# Autodesk Inventor assembly: ASSEMBLY_Main
(part 2 of 4)
157. DIN 125-1 A A 3,2:54 — Mate:569, Mate:570, Insert:151
158. DIN 934 - replaced by DIN EN 24032/28673/28674 M3:16 — Insert:154
159. DIN 125-1 A A 3,2:53 — Mate:575, Mate:576, Insert:154
160. DIN 912 - replaced by DIN EN ISO 4762 M3 x 16:5 — Insert:150
161. DIN 125-1 A A 3,2:52 — Mate:567, Mate:568, Insert:150
162. DIN 934 - replaced by DIN EN 24032/28673/28674 M3:15 — Insert:149
163. DIN 125-1 A A 3,2:51 — Mate:565, Mate:566, Insert:149
164. DIN 912 - replaced by DIN EN ISO 4762 M3 x 10:4 — Insert:147
165. DIN 125-1 A A 3,2:50 — Mate:561, Mate:562, Insert:147
166. DIN 934 - replaced by DIN EN 24032/28673/28674 M3:14 — Insert:148
167. DIN 125-1 A A 3,2:49 — Mate:563, Mate:564, Insert:148
168. DIN 125-1 A A 5,3:51 — Mate:481, Mate:482, Insert:107
169. DIN 125-1 A A 5,3:92 — Mate:603, Mate:604, Insert:168
170. DIN 912 - replaced by DIN EN ISO 4762 M5 x 10:29 — Insert:167
171. DIN 125-1 A A 5,3:91 — Mate:601, Mate:602, Insert:167
172. DIN 912 - replaced by DIN EN ISO 4762 M5 x 10:28 — Insert:166
173. DIN 912 - replaced by DIN EN ISO 4762 M5 x 10:27 — Insert:165
174. DIN 912 - replaced by DIN EN ISO 4762 M5 x 10:26 — Insert:164
175. DIN 125-1 A A 5,3:90 — Mate:599, Mate:600, Insert:166
176. DIN 125-1 A A 5,3:89 — Mate:597, Mate:598, Insert:165
177. DIN 125-1 A A 5,3:88 — Mate:595, Mate:596, Insert:164
178. DIN 912 - replaced by DIN EN ISO 4762 M5 x 10:25 — Insert:163
179. DIN 125-1 A A 5,3:87 — Mate:593, Mate:594, Insert:163
180. DIN 912 - replaced by DIN EN ISO 4762 M5 x 8:25 — Insert:162
181. DIN 125-1 A A 5,3:86 — Mate:591, Mate:592, Insert:162
182. DIN 912 - replaced by DIN EN ISO 4762 M5 x 12:12 — Insert:161
183. DIN 125-1 A A 5,3:85 — Mate:589, Mate:590, Insert:161
184. DIN 912 - replaced by DIN EN ISO 4762 M5 x 12:11 — Insert:160
185. DIN 125-1 A A 5,3:84 — Mate:587, Mate:588, Insert:160
186. DIN 912 - replaced by DIN EN ISO 4762 M5 x 8:24 — Insert:159
187. DIN 125-1 A A 5,3:83 — Mate:585, Mate:586, Insert:159
188. DIN 912 - replaced by DIN EN ISO 4762 M5 x 8:23 — Insert:158
189. DIN 125-1 A A 5,3:82 — Mate:583, Mate:584, Insert:158
190. DIN 934 - replaced by DIN EN 24032/28673/28674 M3:19 — Insert:157
191. DIN 934 - replaced by DIN EN 24032/28673/28674 M3:18 — Insert:156
192. DIN 934 - replaced by DIN EN 24032/28673/28674 M3:17 — Insert:155
193. DIN 912 - replaced by DIN EN ISO 4762 M3 x 10:3 — Insert:146
194. DIN 125-1 A A 3,2:48 — Mate:559, Mate:560, Insert:146
195. DIN 934 - replaced by DIN EN 24032/28673/28674 M3:13 — Insert:145
196. DIN 125-1 A A 3,2:47 — Mate:557, Mate:558, Insert:145
197. DIN 912 - replaced by DIN EN ISO 4762 M3 x 10:2 — Insert:143
198. DIN 125-1 A A 3,2:46 — Mate:553, Mate:554, Insert:143
199. DIN 934 - replaced by DIN EN 24032/28673/28674 M3:12 — Insert:144
200. DIN 125-1 A A 3,2:45 — Mate:555, Mate:556, Insert:144
201. DIN 912 - replaced by DIN EN ISO 4762 M3 x 10:1 — Insert:142
202. DIN 125-1 A A 3,2:44 — Mate:551, Mate:552, Insert:142
203. DIN 912 - replaced by DIN EN ISO 4762 M5 x 30:13 — Insert:141
204. DIN 125-1 A A 5,3:81 — Mate:549, Mate:550, Insert:141
205. DIN 912 - replaced by DIN EN ISO 4762 M5 x 8:22 — Insert:140
206. DIN 125-1 A A 5,3:80 — Mate:547, Mate:548, Insert:140
207. DIN 912 - replaced by DIN EN ISO 4762 M5 x 8:21 — Insert:139
208. DIN 125-1 A A 5,3:79 — Mate:545, Mate:546, Insert:139
209. DIN 912 - replaced by DIN EN ISO 4762 M5 x 10:24 — Insert:138
210. DIN 912 - replaced by DIN EN ISO 4762 M5 x 10:23 — Insert:137
211. DIN 912 - replaced by DIN EN ISO 4762 M5 x 10:22 — Insert:136
212. DIN 125-1 A A 5,3:78 — Mate:543, Mate:544, Insert:138
213. DIN 125-1 A A 5,3:77 — Mate:541, Mate:542, Insert:137
214. DIN 125-1 A A 5,3:76 — Mate:539, Mate:540, Insert:136
215. DIN 912 - replaced by DIN EN ISO 4762 M5 x 10:21 — Insert:135
216. DIN 125-1 A A 5,3:75 — Mate:537, Mate:538, Insert:135
217. DIN 912 - replaced by DIN EN ISO 4762 M5 x 10:20 — Insert:134
218. DIN 912 - replaced by DIN EN ISO 4762 M5 x 10:19 — Insert:133
219. DIN 912 - replaced by DIN EN ISO 4762 M5 x 10:18 — Insert:132
220. DIN 125-1 A A 5,3:74 — Mate:535, Mate:536, Insert:134
221. DIN 125-1 A A 5,3:73 — Mate:533, Mate:534, Insert:133
222. DIN 125-1 A A 5,3:72 — Mate:531, Mate:532, Insert:132
223. DIN 912 - replaced by DIN EN ISO 4762 M5 x 10:17 — Insert:131
224. DIN 125-1 A A 5,3:71 — Mate:529, Mate:530, Insert:131
225. DIN 912 - replaced by DIN EN ISO 4762 M5 x 10:16 — Insert:130
226. DIN 125-1 A A 5,3:70 — Mate:527, Mate:528, Insert:130
227. DIN 912 - replaced by DIN EN ISO 4762 M5 x 10:15 — Insert:129
228. DIN 125-1 A A 5,3:69 — Mate:525, Mate:526, Insert:129
229. DIN 912 - replaced by DIN EN ISO 4762 M5 x 10:14 — Insert:128
230. DIN 125-1 A A 5,3:68 — Mate:523, Mate:524, Insert:128
231. DIN 912 - replaced by DIN EN ISO 4762 M5 x 10:13 — Insert:127
232. DIN 125-1 A A 5,3:67 — Mate:521, Mate:522, Insert:127
233. DIN 912 - replaced by DIN EN ISO 4762 M4 x 10:4 — Insert:126
234. DIN 912 - replaced by DIN EN ISO 4762 M4 x 10:3 — Insert:125
235. DIN 912 - replaced by DIN EN ISO 4762 M4 x 10:2 — Insert:124
236. DIN 125-1 A A 4,3:20 — Mate:519, Mate:520, Insert:126
237. DIN 125-1 A A 4,3:19 — Mate:517, Mate:518, Insert:125
238. DIN 125-1 A A 4,3:18 — Mate:515, Mate:516, Insert:124
239. DIN 912 - replaced by DIN EN ISO 4762 M4 x 10:1 — Insert:123
240. DIN 125-1 A A 4,3:17 — Mate:513, Mate:514, Insert:123
241. DIN 912 - replaced by DIN EN ISO 4762 M4 x 8:4 — Insert:122
242. DIN 912 - replaced by DIN EN ISO 4762 M4 x 8:3 — Insert:121
243. DIN 912 - replaced by DIN EN ISO 4762 M4 x 8:2 — Insert:120
244. DIN 125-1 A A 4,3:16 — Mate:511, Mate:512, Insert:122
245. DIN 125-1 A A 4,3:15 — Mate:509, Mate:510, Insert:121
246. DIN 125-1 A A 4,3:14 — Mate:507, Mate:508, Insert:120
247. DIN 912 - replaced by DIN EN ISO 4762 M4 x 8:1 — Insert:119
248. DIN 125-1 A A 4,3:13 — Mate:505, Mate:506, Insert:119
249. DIN 912 - replaced by DIN EN ISO 4762 M5 x 10:12 — Insert:118
250. DIN 125-1 A A 5,3:66 — Mate:503, Mate:504, Insert:118
251. DIN 912 - replaced by DIN EN ISO 4762 M5 x 10:11 — Insert:117
252. DIN 125-1 A A 5,3:65 — Mate:501, Mate:502, Insert:117
253. DIN 912 - replaced by DIN EN ISO 4762 M5 x 10:10 — Insert:116
254. DIN 125-1 A A 5,3:64 — Mate:499, Mate:500, Insert:116
255. DIN 912 - replaced by DIN EN ISO 4762 M5 x 10:9 — Insert:115
256. DIN 125-1 A A 5,3:63 — Mate:497, Mate:498, Insert:115
257. DIN 912 - replaced by DIN EN ISO 4762 M5 x 12:10 — Insert:114
258. DIN 125-1 A A 5,3:62 — Mate:495, Mate:496, Insert:114
259. DIN 912 - replaced by DIN EN ISO 4762 M5 x 12:9 — Insert:113
260. DIN 125-1 A A 5,3:61 — Mate:493, Mate:494, Insert:113
261. DIN 912 - replaced by DIN EN ISO 4762 M5 x 12:8 — Insert:112
262. DIN 125-1 A A 5,3:60 — Mate:491, Mate:492, Insert:112
263. DIN 912 - replaced by DIN EN ISO 4762 M5 x 12:7 — Insert:111
264. DIN 125-1 A A 5,3:59 — Mate:489, Mate:490, Insert:111
265. DIN 912 - replaced by DIN EN ISO 4762 M5 x 10:8 — Insert:110
266. DIN 125-1 A A 5,3:58 — Mate:487, Mate:488, Insert:110
267. DIN 912 - replaced by DIN EN ISO 4762 M5 x 10:7 — Insert:109
268. DIN 125-1 A A 5,3:57 — Mate:485, Mate:486, Insert:109
269. DIN 912 - replaced by DIN EN ISO 4762 M5 x 10:6 — Insert:108
270. DIN 125-1 A A 5,3:52 — Mate:483, Mate:484, Insert:108
271. DIN 912 - replaced by DIN EN ISO 4762 M5 x 10:5 — Insert:107
272. DIN 912 - replaced by DIN EN ISO 4762 M5 x 10:2 — Insert:106
273. DIN 125-1 A A 5,3:50 — Mate:479, Mate:480, Insert:106
274. DIN 912 - replaced by DIN EN ISO 4762 M5 x 10:1 — Insert:105
275. DIN 125-1 A A 5,3:49 — Mate:477, Mate:478, Insert:105
276. DIN 912 - replaced by DIN EN ISO 4762 M5 x 12:5 — Insert:104
277. DIN 125-1 A A 5,3:53 — Mate:475, Mate:476, Insert:104
278. DIN 912 - replaced by DIN EN ISO 4762 M5 x 12:6 — Insert:103
279. DIN 125-1 A A 5,3:54 — Mate:473, Mate:474, Insert:103
280. DIN 912 - replaced by DIN EN ISO 4762 M5 x 10:3 — Insert:102
281. DIN 125-1 A A 5,3:55 — Mate:471, Mate:472, Insert:102
282. DIN 912 - replaced by DIN EN ISO 4762 M5 x 10:4 — Insert:101
283. DIN 125-1 A A 5,3:56 — Mate:469, Mate:470, Insert:101
284. DIN 912 - replaced by DIN EN ISO 4762 M3 x 8:2 — Insert:66
285. DIN 125-1 A A 3,2:17 — Mate:387, Mate:388, Insert:66
286. DIN 912 - replaced by DIN EN ISO 4762 M3 x 8:1 — Insert:65
287. DIN 125-1 A A 3,2:16 — Mate:385, Mate:386, Insert:65
288. DIN 125-1 A A 3,2:30 — Mate:423, Mate:424, Insert:79
289. DIN 125-1 A A 3,2:29 — Mate:421, Mate:422, Insert:78
290. ISO 7380-1 M3 x 20:9 — Insert:76
291. ISO 7380-1 M3 x 20:8 — Insert:75
292. ISO 7380-1 M3 x 20:7 — Insert:74
293. ISO 7380-1 M3 x 20:6 — Insert:73
294. ISO 7380-1 M3 x 20:5 — Insert:72
295. ISO 7380-1 M3 x 20:4 — Insert:71
296. ISO 7380-1 M3 x 20:3 — Insert:70
297. DIN 125-1 A A 3,2:28 — Mate:417, Mate:418, Insert:76
298. DIN 125-1 A A 3,2:27 — Mate:415, Mate:416, Insert:75
299. DIN 125-1 A A 3,2:26 — Mate:413, Mate:414, Insert:74
300. DIN 125-1 A A 3,2:25 — Mate:411, Mate:412, Insert:73
301. DIN 125-1 A A 3,2:24 — Mate:409, Mate:410, Insert:72
302. DIN 125-1 A A 3,2:23 — Mate:407, Mate:408, Insert:71
303. DIN 125-1 A A 3,2:22 — Mate:405, Mate:406, Insert:70
304. DIN 934 - replaced by DIN EN 24032/28673/28674 M3:4 — Insert:77
305. DIN 125-1 A A 3,2:21 — Mate:419, Mate:420, Insert:77
306. ISO 7380-1 M3 x 20:2 — Insert:69
307. DIN 125-1 A A 3,2:20 — Mate:403, Mate:404, Insert:69
308. DIN 7991 M3x8:2 — Mate:402
309. DIN 7991 M3x8:1 — Mate:401
310. DIN 912 - replaced by DIN EN ISO 4762 M3 x 8:4 — Insert:68
311. DIN 125-1 A A 3,2:19 — Mate:393, Mate:394, Insert:68
312. DIN 912 - replaced by DIN EN ISO 4762 M3 x 8:3 — Insert:67
313. DIN 125-1 A A 3,2:18 — Mate:391, Mate:392, Insert:67
314. DIN 125-1 A A 3,2:43 — Mate:451, Mate:452, Insert:92
315. DIN 125-1 A A 3,2:42 — Mate:449, Mate:450, Insert:91
316. DIN 125-1 A A 3,2:41 — Mate:447, Mate:448, Insert:90
317. DIN 125-1 A A 3,2:40 — Mate:445, Mate:446, Insert:89
318. DIN 125-1 A A 3,2:39 — Mate:443, Mate:444, Insert:88
319. DIN 125-1 A A 3,2:38 — Mate:441, Mate:442, Insert:87
320. DIN 125-1 A A 3,2:37 — Mate:439, Mate:440, Insert:86
321. DIN 912 - replaced by DIN EN ISO 4762 M3 x 8:5 — Insert:85
322. DIN 125-1 A A 3,2:36 — Mate:437, Mate:438, Insert:85
323. DIN 934 - replaced by DIN EN 24032/28673/28674 M3:11 — Insert:84
324. DIN 934 - replaced by DIN EN 24032/28673/28674 M3:10 — Insert:83
325. DIN 934 - replaced by DIN EN 24032/28673/28674 M3:9 — Insert:82
326. DIN 934 - replaced by DIN EN 24032/28673/28674 M3:8 — Insert:81
327. DIN 934 - replaced by DIN EN 24032/28673/28674 M3:7 — Insert:80
328. DIN 934 - replaced by DIN EN 24032/28673/28674 M3:6 — Insert:79
329. DIN 934 - replaced by DIN EN 24032/28673/28674 M3:5 — Insert:78
330. DIN 125-1 A A 3,2:35 — Mate:433, Mate:434, Insert:84
331. DIN 125-1 A A 3,2:34 — Mate:431, Mate:432, Insert:83
332. DIN 125-1 A A 3,2:33 — Mate:429, Mate:430, Insert:82
333. DIN 125-1 A A 3,2:32 — Mate:427, Mate:428, Insert:81
334. DIN 125-1 A A 3,2:31 — Mate:425, Mate:426, Insert:80
335. DIN 934 - replaced by DIN EN 24032/28673/28674 M4:6 — Insert:100
336. DIN 934 - replaced by DIN EN 24032/28673/28674 M4:5 — Insert:99
337. DIN 934 - replaced by DIN EN 24032/28673/28674 M4:4 — Insert:98
338. DIN 125-1 A A 4,3:12 — Mate:467, Mate:468, Insert:100
339. DIN 125-1 A A 4,3:11 — Mate:465, Mate:466, Insert:99
340. DIN 125-1 A A 4,3:10 — Mate:463, Mate:464, Insert:98
341. DIN 912 - replaced by DIN EN ISO 4762 M4 x 40:4 — Insert:96
342. DIN 912 - replaced by DIN EN ISO 4762 M4 x 40:3 — Insert:95
343. DIN 912 - replaced by DIN EN ISO 4762 M4 x 40:2 — Insert:94
344. DIN 125-1 A A 4,3:9 — Mate:459, Mate:460, Insert:96
345. DIN 125-1 A A 4,3:8 — Mate:457, Mate:458, Insert:95
346. DIN 125-1 A A 4,3:7 — Mate:455, Mate:456, Insert:94
347. DIN 934 - replaced by DIN EN 24032/28673/28674 M4:3 — Insert:97
348. DIN 125-1 A A 4,3:6 — Mate:461, Mate:462, Insert:97
349. DIN 912 - replaced by DIN EN ISO 4762 M4 x 40:1 — Insert:93
350. DIN 125-1 A A 4,3:5 — Mate:453, Mate:454, Insert:93
351. DIN 912 - replaced by DIN EN ISO 4762 M3 x 8:12 — Insert:92
352. DIN 912 - replaced by DIN EN ISO 4762 M3 x 8:11 — Insert:91
353. DIN 912 - replaced by DIN EN ISO 4762 M3 x 8:10 — Insert:90
354. DIN 912 - replaced by DIN EN ISO 4762 M3 x 8:9 — Insert:89
355. DIN 912 - replaced by DIN EN ISO 4762 M3 x 8:8 — Insert:88
356. DIN 912 - replaced by DIN EN ISO 4762 M3 x 8:7 — Insert:87
357. DIN 912 - replaced by DIN EN ISO 4762 M3 x 8:6 — Insert:86
358. DIN 912 - replaced by DIN EN ISO 4762 M5 x 8:5 — Insert:45
359. DIN 912 - replaced by DIN EN ISO 4762 M5 x 8:4 — Insert:44
360. DIN 912 - replaced by DIN EN ISO 4762 M5 x 8:3 — Insert:43
361. DIN 912 - replaced by DIN EN ISO 4762 M5 x 8:2 — Insert:42
362. DIN 125-1 A A 5,3:29 — Mate:336, Mate:337, Insert:45
363. DIN 125-1 A A 5,3:28 — Mate:334, Mate:335, Insert:44
364. DIN 125-1 A A 5,3:27 — Mate:332, Mate:333, Insert:43
365. DIN 125-1 A A 5,3:26 — Mate:330, Mate:331, Insert:42
366. DIN 912 - replaced by DIN EN ISO 4762 M5 x 8:1 — Insert:41
367. DIN 125-1 A A 5,3:25 — Mate:328, Mate:329, Insert:41
368. DIN 934 - replaced by DIN EN 24032/28673/28674 M5:4 — Insert:40
369. DIN 125-1 A A 5,3:24 — Mate:326, Mate:327, Insert:40
370. DIN 912 - replaced by DIN EN ISO 4762 M5 x 25:4 — Insert:38
371. DIN 125-1 A A 5,3:23 — Mate:322, Mate:323, Insert:38
372. DIN 934 - replaced by DIN EN 24032/28673/28674 M5:3 — Insert:39
373. DIN 125-1 A A 5,3:22 — Mate:324, Mate:325, Insert:39
374. DIN 912 - replaced by DIN EN ISO 4762 M5 x 25:3 — Insert:37
375. DIN 125-1 A A 5,3:21 — Mate:320, Mate:321, Insert:37
376. DIN 934 - replaced by DIN EN 24032/28673/28674 M5:2 — Insert:36
377. DIN 125-1 A A 5,3:20 — Mate:318, Mate:319, Insert:36
378. DIN 912 - replaced by DIN EN ISO 4762 M5 x 25:2 — Insert:34
379. DIN 125-1 A A 5,3:19 — Mate:314, Mate:315, Insert:34
380. DIN 934 - replaced by DIN EN 24032/28673/28674 M5:1 — Insert:35
381. DIN 125-1 A A 5,3:18 — Mate:316, Mate:317, Insert:35
382. DIN 912 - replaced by DIN EN ISO 4762 M5 x 25:1 — Insert:33
383. DIN 125-1 A A 5,3:17 — Mate:312, Mate:313, Insert:33
384. DIN 912 - replaced by DIN EN ISO 4762 M5 x 8:10 — Insert:50
385. DIN 912 - replaced by DIN EN ISO 4762 M5 x 8:9 — Insert:49
386. DIN 912 - replaced by DIN EN ISO 4762 M5 x 8:8 — Insert:48
387. DIN 912 - replaced by DIN EN ISO 4762 M5 x 8:7 — Insert:47
388. DIN 125-1 A A 5,3:34 — Insert:50
389. DIN 125-1 A A 5,3:33 — Insert:49
390. DIN 125-1 A A 5,3:32 — Insert:48
391. DIN 125-1 A A 5,3:31 — Insert:47
392. DIN 912 - replaced by DIN EN ISO 4762 M5 x 8:6 — Insert:46
393. DIN 125-1 A A 5,3:30 — Insert:46
394. DIN 912 - replaced by DIN EN ISO 4762 M5 x 8:15 — Insert:55
395. DIN 912 - replaced by DIN EN ISO 4762 M5 x 8:14 — Insert:54
396. DIN 912 - replaced by DIN EN ISO 4762 M5 x 8:13 — Insert:53
397. DIN 912 - replaced by DIN EN ISO 4762 M5 x 8:12 — Insert:52
398. DIN 125-1 A A 5,3:39 — Insert:55
399. DIN 125-1 A A 5,3:38 — Insert:54
400. DIN 125-1 A A 5,3:37 — Insert:53
401. DIN 125-1 A A 5,3:36 — Insert:52
402. DIN 912 - replaced by DIN EN ISO 4762 M5 x 8:11 — Insert:51
403. DIN 125-1 A A 5,3:35 — Insert:51
404. DIN 912 - replaced by DIN EN ISO 4762 M5 x 12:4 — Insert:64
405. DIN 912 - replaced by DIN EN ISO 4762 M5 x 12:3 — Insert:63
406. DIN 912 - replaced by DIN EN ISO 4762 M5 x 12:2 — Insert:62
407. DIN 125-1 A A 5,3:48 — Mate:371, Mate:372, Insert:64
408. DIN 125-1 A A 5,3:47 — Mate:369, Mate:370, Insert:63
409. DIN 125-1 A A 5,3:46 — Mate:367, Mate:368, Insert:62
410. DIN 912 - replaced by DIN EN ISO 4762 M5 x 12:1 — Insert:61
411. DIN 125-1 A A 5,3:45 — Mate:365, Mate:366, Insert:61
412. DIN 912 - replaced by DIN EN ISO 4762 M5 x 8:20 — Insert:60
413. DIN 912 - replaced by DIN EN ISO 4762 M5 x 8:19 — Insert:59
414. DIN 912 - replaced by DIN EN ISO 4762 M5 x 8:18 — Insert:58
415. DIN 912 - replaced by DIN EN ISO 4762 M5 x 8:17 — Insert:57
416. DIN 125-1 A A 5,3:44 — Insert:60
417. DIN 125-1 A A 5,3:43 — Insert:59
418. DIN 125-1 A A 5,3:42 — Insert:58
419. DIN 125-1 A A 5,3:41 — Insert:57
420. DIN 912 - replaced by DIN EN ISO 4762 M5 x 8:16 — Insert:56
421. DIN 125-1 A A 5,3:40 — Insert:56
422. DIN 934 - replaced by DIN EN 24032/28673/28674 M4:2 — Insert:31
423. DIN 125-1 A A 4,3:4 — Mate:304, Mate:305, Insert:31
424. DIN 912 - replaced by DIN EN ISO 4762 M4 x 30:2 — Insert:29
425. DIN 125-1 A A 4,3:3 — Mate:300, Mate:301, Insert:29
426. DIN 934 - replaced by DIN EN 24032/28673/28674 M4:1 — Insert:30
427. DIN 125-1 A A 4,3:2 — Mate:302, Mate:303, Insert:30
428. DIN 912 - replaced by DIN EN ISO 4762 M4 x 30:1 — Insert:28
429. DIN 125-1 A A 4,3:1 — Mate:298, Mate:299, Insert:28
430. DIN 934 - replaced by DIN EN 24032/28673/28674 M3:3 — Insert:27
431. DIN 125-1 A A 3,2:11 — Mate:296, Mate:297, Insert:27
432. DIN 912 - replaced by DIN EN ISO 4762 M3 x 20:1 — Insert:26
433. DIN 125-1 A A 3,2:10 — Mate:294, Mate:295, Insert:26
434. DIN 934 - replaced by DIN EN 24032/28673/28674 M3:2 — Insert:25
435. DIN 125-1 A A 3,2:9 — Mate:292, Mate:293, Insert:25
436. ISO 7380-1 M3 x 20:1 — Insert:24
437. DIN 125-1 A A 3,2:8 — Mate:290, Mate:291, Insert:24
438. DIN 934 - replaced by DIN EN 24032/28673/28674 M3:1 — Insert:23
439. DIN 125-1 A A 3,2:7 — Mate:288, Mate:289, Insert:23
440. ISO 7380-1 M3 x 30:1 — Insert:22
441. DIN 125-1 A A 3,2:6 — Mate:286, Mate:287, Insert:22
442. ISO 7380-1 M3 x 12:5 — Insert:21
443. ISO 7380-1 M3 x 12:4 — Insert:20
444. ISO 7380-1 M3 x 12:3 — Insert:19
445. ISO 7380-1 M3 x 12:2 — Insert:18
446. DIN 125-1 A A 3,2:5 — Mate:284, Mate:285, Insert:21
447. DIN 125-1 A A 3,2:4 — Mate:282, Mate:283, Insert:20
448. DIN 125-1 A A 3,2:3 — Mate:280, Mate:281, Insert:19
449. DIN 125-1 A A 3,2:2 — Mate:278, Mate:279, Insert:18
450. ISO 7380-1 M3 x 12:1 — Insert:17
451. DIN 125-1 A A 3,2:1 — Mate:276, Mate:277, Insert:17
452. DIN 912 - replaced by DIN EN ISO 4762 M5 x 50:4 — Insert:16
453. DIN 912 - replaced by DIN EN ISO 4762 M5 x 50:3 — Insert:15
454. DIN 912 - replaced by DIN EN ISO 4762 M5 x 50:2 — Insert:14
455. DIN 125-1 A A 5,3:16 — Mate:274, Mate:275, Insert:16
456. DIN 125-1 A A 5,3:15 — Mate:272, Mate:273, Insert:15
457. DIN 125-1 A A 5,3:14 — Mate:270, Mate:271, Insert:14
458. DIN 912 - replaced by DIN EN ISO 4762 M5 x 50:1 — Insert:13
459. DIN 125-1 A A 5,3:13 — Mate:268, Mate:269, Insert:13
460. DIN 912 - replaced by DIN EN ISO 4762 M5 x 30:12 — Insert:12
461. DIN 912 - replaced by DIN EN ISO 4762 M5 x 30:11 — Insert:11
462. DIN 912 - replaced by DIN EN ISO 4762 M5 x 30:10 — Insert:10
463. DIN 912 - replaced by DIN EN ISO 4762 M5 x 30:9 — Insert:9
464. DIN 912 - replaced by DIN EN ISO 4762 M5 x 30:8 — Insert:8
465. DIN 912 - replaced by DIN EN ISO 4762 M5 x 30:7 — Insert:7
466. DIN 912 - replaced by DIN EN ISO 4762 M5 x 30:6 — Insert:6
467. DIN 912 - replaced by DIN EN ISO 4762 M5 x 30:5 — Insert:5
468. DIN 912 - replaced by DIN EN ISO 4762 M5 x 30:4 — Insert:4
469. DIN 912 - replaced by DIN EN ISO 4762 M5 x 30:3 — Insert:3
470. DIN 912 - replaced by DIN EN ISO 4762 M5 x 30:2 — Insert:2
471. DIN 125-1 A A 5,3:12 — Mate:266, Mate:267, Insert:12
472. DIN 125-1 A A 5,3:11 — Mate:264, Mate:265, Insert:11
473. DIN 125-1 A A 5,3:10 — Mate:262, Mate:263, Insert:10
474. DIN 125-1 A A 5,3:9 — Mate:260, Mate:261, Insert:9
475. DIN 125-1 A A 5,3:8 — Mate:258, Mate:259, Insert:8
476. DIN 125-1 A A 5,3:7 — Mate:256, Mate:257, Insert:7
477. DIN 125-1 A A 5,3:6 — Mate:254, Mate:255, Insert:6
478. DIN 125-1 A A 5,3:5 — Mate:252, Mate:253, Insert:5
479. DIN 125-1 A A 5,3:4 — Mate:250, Mate:251, Insert:4
480. DIN 125-1 A A 5,3:3 — Mate:248, Mate:249, Insert:3
481. DIN 125-1 A A 5,3:2 — Mate:246, Mate:247, Insert:2
482. DIN 912 - replaced by DIN EN ISO 4762 M5 x 30:1 — Insert:1
483. DIN 125-1 A A 5,3:1 — Mate:244, Mate:245, Insert:1
484. ISO 10642 M4x20:1 — Mate:641, Mate:642
485. DIN 934 - replaced by DIN EN 24032/28673/28674 M4:8 — Insert:172
486. DIN 934 - replaced by DIN EN 24032/28673/28674 M4:7 — Insert:171
487. ISO 10642 M4x20:2
488. DIN 934 - replaced by DIN EN 24032/28673/28674 M4:9
489. DIN 934 - replaced by DIN EN 24032/28673/28674 M4:10
490. ISO 10642 M4x20:3
491. DIN 934 - replaced by DIN EN 24032/28673/28674 M4:11
492. DIN 934 - replaced by DIN EN 24032/28673/28674 M4:12
493. ISO 10642 M4x20:4
494. DIN 934 - replaced by DIN EN 24032/28673/28674 M4:13
495. DIN 934 - replaced by DIN EN 24032/28673/28674 M4:14
496. DIN 912 - replaced by DIN EN ISO 4762 M3 x 16:1 — Insert:32, Mate:310
497. DIN 125-1 A A 3,2:12 — Mate:308, Mate:309, Insert:32
498. COTS_GENERIC_20x20_M3_Nut:1 — Mate:306, Mate:307, Mate:310
499. DIN 912 - replaced by DIN EN ISO 4762 M3 x 16:2
500. DIN 125-1 A A 3,2:13
501. COTS_GENERIC_20x20_M3_Nut:2
502. DIN 912 - replaced by DIN EN ISO 4762 M3 x 16:3
503. DIN 125-1 A A 3,2:14
504. COTS_GENERIC_20x20_M3_Nut:3
505. DIN 912 - replaced by DIN EN ISO 4762 M3 x 16:4
506. DIN 125-1 A A 3,2:15
507. COTS_GENERIC_20x20_M3_Nut:4
## Component patterns: (2 elements), (4 elements, first: ISO 10642 M4x20:1 + DIN 934 - replaced by DIN EN 24032/28673/28674 M4:8 + DIN 934 - replaced by DIN EN 24032/28673/28674 M4:7), (2 elements, first: DIN 912 - replaced by DIN EN ISO 4762 M3 x 16:1 + DIN 125-1 A A 3,2:12 + COTS_GENERIC_20x20_M3_Nut:1), Component Pattern 1:2 (2 elements)
## Relationships (862: Mate 549, Insert 172, Flush 139, Angle 2)
- Zestawiający:7 [Mate]: COTS_GENERIC_20x40mm_alu_extrusion_460mm:1 ↔ COTS_GENERIC_20x40mm_alu_extrusion_560mm:1
- Równoległy:13 [Flush]: COTS_GENERIC_20x40mm_alu_extrusion_460mm:1 ↔ COTS_GENERIC_20x40mm_alu_extrusion_560mm:1
- Równoległy:14 [Flush]: COTS_GENERIC_20x40mm_alu_extrusion_460mm:1 ↔ COTS_GENERIC_20x40mm_alu_extrusion_560mm:1
- Zestawiający:8 [Mate]: COTS_GENERIC_20x40mm_alu_extrusion_460mm:2 ↔ COTS_GENERIC_20x40mm_alu_extrusion_560mm:1
- Równoległy:15 [Flush]: COTS_GENERIC_20x40mm_alu_extrusion_460mm:2 ↔ COTS_GENERIC_20x40mm_alu_extrusion_560mm:1
- Równoległy:16 [Flush]: COTS_GENERIC_20x40mm_alu_extrusion_460mm:2 ↔ COTS_GENERIC_20x40mm_alu_extrusion_560mm:1
- Zestawiający:9 [Mate]: COTS_GENERIC_20x40mm_alu_extrusion_460mm:1 ↔ COTS_GENERIC_20x40mm_alu_extrusion_560mm:3
- Równoległy:17 [Flush]: COTS_GENERIC_20x40mm_alu_extrusion_460mm:1 ↔ COTS_GENERIC_20x40mm_alu_extrusion_560mm:3
- Równoległy:18 [Flush]: COTS_GENERIC_20x40mm_alu_extrusion_460mm:1 ↔ COTS_GENERIC_20x40mm_alu_extrusion_560mm:3
- Zestawiający:10 [Mate]: COTS_GENERIC_20x40mm_alu_extrusion_460mm:1 ↔ COTS_GENERIC_20x40mm_alu_extrusion_460mm:3
- Równoległy:19 [Flush]: COTS_GENERIC_20x40mm_alu_extrusion_460mm:1 ↔ COTS_GENERIC_20x40mm_alu_extrusion_460mm:3
- Zestawiający:11 [Mate]: COTS_GENERIC_20x40mm_alu_extrusion_460mm:2 ↔ COTS_GENERIC_20x40mm_alu_extrusion_460mm:4
- Równoległy:20 [Flush]: COTS_GENERIC_20x40mm_alu_extrusion_460mm:2 ↔ COTS_GENERIC_20x40mm_alu_extrusion_460mm:4
- Zestawiający:12 [Mate]: COTS_GENERIC_20x40mm_alu_extrusion_460mm:3 ↔ COTS_GENERIC_20x40mm_alu_extrusion_560mm:2
- Równoległy:21 [Flush]: COTS_GENERIC_20x40mm_alu_extrusion_460mm:3 ↔ COTS_GENERIC_20x40mm_alu_extrusion_560mm:2
- Równoległy:22 [Flush]: COTS_GENERIC_20x40mm_alu_extrusion_460mm:3 ↔ COTS_GENERIC_20x40mm_alu_extrusion_560mm:2
- Równoległy:23 [Flush]: COTS_GENERIC_20x40mm_alu_extrusion_460mm:4 ↔ COTS_GENERIC_20x40mm_alu_extrusion_560mm:2
- Równoległy:24 [Flush]: COTS_GENERIC_20x40mm_alu_extrusion_460mm:4 ↔ COTS_GENERIC_20x40mm_alu_extrusion_560mm:2
- Równoległy:25 [Flush] (156.5 mm): COTS_GENERIC_20x40mm_alu_extrusion_460mm:1 ↔ COTS_GENERIC_20x40mm_alu_extrusion_460mm:3
- Zestawiający:13 [Mate]: COTS_GENERIC_20x40mm_alu_extrusion_460mm:3 ↔ LC_ALU_3mm_Top_Beam_Mounting_Bracket:1
- Zestawiający:14 [Mate]: COTS_GENERIC_20x40mm_alu_extrusion_560mm:2 ↔ LC_ALU_3mm_Top_Beam_Mounting_Bracket:2
- Zestawiający:15 [Mate]: COTS_GENERIC_20x40mm_alu_extrusion_560mm:2 ↔ LC_ALU_3mm_Top_Beam_Mounting_Bracket:3
- Zestawiający:16 [Mate]: COTS_GENERIC_20x40mm_alu_extrusion_460mm:4 ↔ LC_ALU_3mm_Top_Beam_Mounting_Bracket:4
- Równoległy:26 [Flush]: COTS_GENERIC_20x40mm_alu_extrusion_460mm:3 ↔ LC_ALU_3mm_Top_Beam_Mounting_Bracket:2
- Równoległy:27 [Flush]: COTS_GENERIC_20x40mm_alu_extrusion_560mm:2 ↔ LC_ALU_3mm_Top_Beam_Mounting_Bracket:2
- Równoległy:28 [Flush]: COTS_GENERIC_20x40mm_alu_extrusion_460mm:3 ↔ LC_ALU_3mm_Top_Beam_Mounting_Bracket:1
- Równoległy:29 [Flush]: COTS_GENERIC_20x40mm_alu_extrusion_560mm:2 ↔ LC_ALU_3mm_Top_Beam_Mounting_Bracket:1
- Równoległy:30 [Flush]: COTS_GENERIC_20x40mm_alu_extrusion_560mm:2 ↔ LC_ALU_3mm_Top_Beam_Mounting_Bracket:3
- Równoległy:31 [Flush]: COTS_GENERIC_20x40mm_alu_extrusion_460mm:4 ↔ LC_ALU_3mm_Top_Beam_Mounting_Bracket:3
- Równoległy:33 [Flush]: COTS_GENERIC_20x40mm_alu_extrusion_560mm:2 ↔ LC_ALU_3mm_Top_Beam_Mounting_Bracket:4
- Zestawiający:17 [Mate]: COTS_GENERIC_20x40mm_alu_extrusion_560mm:2 ↔ COTS_GENERIC_20x40_Alu_Extrusion_Endcap:2
- Zestawiający:18 [Mate]: COTS_GENERIC_20x40mm_alu_extrusion_560mm:3 ↔ COTS_GENERIC_20x40_Alu_Extrusion_Endcap:1
- Zestawiający:19 [Mate]: COTS_GENERIC_20x40mm_alu_extrusion_560mm:1 ↔ COTS_GENERIC_20x40_Alu_Extrusion_Endcap:3
- Zestawiający:20 [Mate]: COTS_GENERIC_20x40mm_alu_extrusion_560mm:2 ↔ COTS_GENERIC_20x40_Alu_Extrusion_Endcap:4
- Zestawiający:21 [Mate]: COTS_GENERIC_20x40mm_alu_extrusion_560mm:1 ↔ COTS_GENERIC_20x40_Alu_Extrusion_Endcap:5
- Zestawiający:22 [Mate]: COTS_GENERIC_20x40mm_alu_extrusion_560mm:3 ↔ COTS_GENERIC_20x40_Alu_Extrusion_Endcap:6
- Równoległy:34 [Flush]: COTS_GENERIC_20x40mm_alu_extrusion_560mm:1 ↔ COTS_GENERIC_20x40_Alu_Extrusion_Endcap:5
- Równoległy:35 [Flush]: COTS_GENERIC_20x40mm_alu_extrusion_560mm:1 ↔ COTS_GENERIC_20x40_Alu_Extrusion_Endcap:5
- Równoległy:36 [Flush]: COTS_GENERIC_20x40mm_alu_extrusion_560mm:3 ↔ COTS_GENERIC_20x40_Alu_Extrusion_Endcap:6
- Równoległy:37 [Flush]: COTS_GENERIC_20x40mm_alu_extrusion_560mm:3 ↔ COTS_GENERIC_20x40_Alu_Extrusion_Endcap:6
- Równoległy:38 [Flush]: COTS_GENERIC_20x40mm_alu_extrusion_560mm:2 ↔ COTS_GENERIC_20x40_Alu_Extrusion_Endcap:4
- Równoległy:39 [Flush]: COTS_GENERIC_20x40mm_alu_extrusion_560mm:2 ↔ COTS_GENERIC_20x40_Alu_Extrusion_Endcap:4
- Równoległy:40 [Flush]: COTS_GENERIC_20x40mm_alu_extrusion_560mm:2 ↔ COTS_GENERIC_20x40_Alu_Extrusion_Endcap:2
- Równoległy:41 [Flush]: COTS_GENERIC_20x40mm_alu_extrusion_560mm:2 ↔ COTS_GENERIC_20x40_Alu_Extrusion_Endcap:2
- Równoległy:42 [Flush]: COTS_GENERIC_20x40mm_alu_extrusion_460mm:4 ↔ LC_ALU_3mm_Top_Beam_Mounting_Bracket:4
- Równoległy:43 [Flush]: COTS_GENERIC_20x40mm_alu_extrusion_560mm:1 ↔ COTS_GENERIC_20x40_Alu_Extrusion_Endcap:3
- Równoległy:44 [Flush]: COTS_GENERIC_20x40mm_alu_extrusion_560mm:1 ↔ COTS_GENERIC_20x40_Alu_Extrusion_Endcap:3
- Równoległy:45 [Flush]: COTS_GENERIC_20x40mm_alu_extrusion_560mm:3 ↔ COTS_GENERIC_20x40_Alu_Extrusion_Endcap:1
- Równoległy:46 [Flush]: COTS_GENERIC_20x40mm_alu_extrusion_560mm:3 ↔ COTS_GENERIC_20x40_Alu_Extrusion_Endcap:1
- Zestawiający:24 [Mate]: COTS_GENERIC_20x40mm_alu_extrusion_460mm:3 ↔ COTS_GENERIC_20x20mm_Angle_Bracket:2
- Zestawiający:26 [Mate]: COTS_GENERIC_20x40mm_alu_extrusion_460mm:4 ↔ COTS_GENERIC_20x20mm_Angle_Bracket:5
- Równoległy:47 [Flush]: COTS_GENERIC_20x40mm_alu_extrusion_460mm:2 ↔ COTS_GENERIC_20x20mm_Angle_Bracket:5
- Równoległy:48 [Flush]: COTS_GENERIC_20x40mm_alu_extrusion_460mm:1 ↔ COTS_GENERIC_20x20mm_Angle_Bracket:2
- Zestawiający:27 [Mate]: COTS_GENERIC_20x40mm_alu_extrusion_460mm:2 ↔ COTS_GENERIC_20x20mm_Angle_Bracket:8
- Zestawiający:28 [Mate]: COTS_GENERIC_20x40mm_alu_extrusion_460mm:1 ↔ COTS_GENERIC_20x20mm_Angle_Bracket:3
- Zestawiający:29 [Mate]: COTS_GENERIC_20x40mm_alu_extrusion_460mm:4 ↔ COTS_GENERIC_20x20mm_Angle_Bracket:8
- Zestawiający:30 [Mate]: COTS_GENERIC_20x40mm_alu_extrusion_460mm:3 ↔ COTS_GENERIC_20x20mm_Angle_Bracket:3
- Równoległy:49 [Flush]: COTS_GENERIC_20x40mm_alu_extrusion_460mm:3 ↔ COTS_GENERIC_20x20mm_Angle_Bracket:3
- Równoległy:50 [Flush]: COTS_GENERIC_20x40mm_alu_extrusion_460mm:4 ↔ COTS_GENERIC_20x20mm_Angle_Bracket:8
- Zestawiający:31 [Mate]: COTS_GENERIC_20x40mm_alu_extrusion_460mm:2 ↔ COTS_GENERIC_20x20mm_Angle_Bracket:6
- Zestawiający:32 [Mate]: COTS_GENERIC_20x40mm_alu_extrusion_460mm:1 ↔ COTS_GENERIC_20x20mm_Angle_Bracket:7
- Zestawiający:33 [Mate]: COTS_GENERIC_20x40mm_alu_extrusion_460mm:2 ↔ COTS_GENERIC_20x20mm_Angle_Bracket:1
- Zestawiający:34 [Mate]: COTS_GENERIC_20x40mm_alu_extrusion_460mm:1 ↔ COTS_GENERIC_20x20mm_Angle_Bracket:4
- Zestawiający:35 [Mate]: COTS_GENERIC_20x40mm_alu_extrusion_560mm:1 ↔ COTS_GENERIC_20x20mm_Angle_Bracket:7
- Zestawiający:36 [Mate]: COTS_GENERIC_20x40mm_alu_extrusion_560mm:1 ↔ COTS_GENERIC_20x20mm_Angle_Bracket:6
- Równoległy:51 [Flush]: COTS_GENERIC_20x40mm_alu_extrusion_460mm:2 ↔ COTS_GENERIC_20x20mm_Angle_Bracket:6
- Równoległy:52 [Flush]: COTS_GENERIC_20x40mm_alu_extrusion_460mm:1 ↔ COTS_GENERIC_20x20mm_Angle_Bracket:7
- Zestawiający:37 [Mate]: COTS_GENERIC_20x40mm_alu_extrusion_560mm:3 ↔ COTS_GENERIC_20x20mm_Angle_Bracket:1
- Zestawiający:38 [Mate]: COTS_GENERIC_20x40mm_alu_extrusion_560mm:3 ↔ COTS_GENERIC_20x20mm_Angle_Bracket:4
- Równoległy:53 [Flush]: COTS_GENERIC_20x40mm_alu_extrusion_460mm:1 ↔ COTS_GENERIC_20x20mm_Angle_Bracket:4
- Równoległy:54 [Flush]: COTS_GENERIC_20x40mm_alu_extrusion_460mm:2 ↔ COTS_GENERIC_20x20mm_Angle_Bracket:1
- Zestawiający:39 [Mate]: COTS_GENERIC_20x40mm_alu_extrusion_460mm:2 ↔ COTS_GENERIC_SK12_Linear_Rail_Mount:2
- Zestawiający:40 [Mate]: COTS_GENERIC_20x40mm_alu_extrusion_460mm:1 ↔ COTS_GENERIC_SK12_Linear_Rail_Mount:1
- Równoległy:55 [Flush] (3 mm): COTS_GENERIC_20x40mm_alu_extrusion_460mm:1 ↔ COTS_GENERIC_SK12_Linear_Rail_Mount:1
- Równoległy:56 [Flush] (3 mm): COTS_GENERIC_20x40mm_alu_extrusion_460mm:2 ↔ COTS_GENERIC_SK12_Linear_Rail_Mount:2
- Zestawiający:41 [Mate]: COTS_GENERIC_20x40mm_alu_extrusion_560mm:2 ↔ COTS_GENERIC_SHF12_Linear_Rail_Mount:1
- Zestawiający:42 [Mate]: COTS_GENERIC_20x40mm_alu_extrusion_560mm:2 ↔ COTS_GENERIC_SHF12_Linear_Rail_Mount:2
- Równoległy:57 [Flush] (-1 mm): COTS_GENERIC_20x40mm_alu_extrusion_460mm:3 ↔ COTS_GENERIC_SK12_Linear_Rail_Mount:1
- Równoległy:58 [Flush] (1 mm): COTS_GENERIC_20x40mm_alu_extrusion_460mm:4 ↔ COTS_GENERIC_SK12_Linear_Rail_Mount:2
- Zestawiający:43 [Mate]: COTS_GENERIC_SK12_Linear_Rail_Mount:2 ↔ CUT_STEEL_12mmx495mm_Linear_Shaft:2
- Zestawiający:44 [Mate]: COTS_GENERIC_SHF12_Linear_Rail_Mount:1 ↔ CUT_STEEL_12mmx495mm_Linear_Shaft:2
- Zestawiający:45 [Mate]: COTS_GENERIC_SK12_Linear_Rail_Mount:1 ↔ CUT_STEEL_12mmx495mm_Linear_Shaft:1
- Zestawiający:46 [Mate]: COTS_GENERIC_SHF12_Linear_Rail_Mount:2 ↔ CUT_STEEL_12mmx495mm_Linear_Shaft:1
- Zestawiający:47 [Mate]: COTS_GENERIC_20x40mm_alu_extrusion_560mm:2 ↔ CUT_STEEL_12mmx495mm_Linear_Shaft:1
- Zestawiający:48 [Mate]: COTS_GENERIC_20x40mm_alu_extrusion_560mm:2 ↔ CUT_STEEL_12mmx495mm_Linear_Shaft:2
- Zestawiający:49 [Mate]: CUT_STEEL_12mmx495mm_Linear_Shaft:1 ↔ COTS_GENERIC_SMA12GUU_Linear_Bearing_Block:4
- Zestawiający:50 [Mate]: CUT_STEEL_12mmx495mm_Linear_Shaft:1 ↔ COTS_GENERIC_SMA12GUU_Linear_Bearing_Block:2
- Zestawiający:51 [Mate]: CUT_STEEL_12mmx495mm_Linear_Shaft:2 ↔ COTS_GENERIC_SMA12GUU_Linear_Bearing_Block:3
- Zestawiający:52 [Mate]: CUT_STEEL_12mmx495mm_Linear_Shaft:2 ↔ COTS_GENERIC_SMA12GUU_Linear_Bearing_Block:1
- Zestawiający:53 [Mate]: COTS_GENERIC_20x40mm_alu_extrusion_560mm:1 ↔ COTS_GENERIC_SHF10_Linear_Rail_Mount:2
- Zestawiający:54 [Mate]: COTS_GENERIC_20x40mm_alu_extrusion_560mm:1 ↔ COTS_GENERIC_SHF10_Linear_Rail_Mount:1
- Zestawiający:55 [Mate]: COTS_GENERIC_20x40mm_alu_extrusion_560mm:3 ↔ COTS_GENERIC_SHF10_Linear_Rail_Mount:3
- Zestawiający:56 [Mate]: COTS_GENERIC_20x40mm_alu_extrusion_560mm:3 ↔ COTS_GENERIC_SHF10_Linear_Rail_Mount:4
- Zestawiający:57 [Mate]: COTS_GENERIC_SHF10_Linear_Rail_Mount:2 ↔ CUT_STEEL_10mmx457mm_Linear_Shaft:1
- Zestawiający:58 [Mate]: COTS_GENERIC_SHF10_Linear_Rail_Mount:1 ↔ CUT_STEEL_10mmx457mm_Linear_Shaft:2
- Równoległy:59 [Flush] (-3.5 mm): COTS_GENERIC_20x40mm_alu_extrusion_560mm:1 ↔ COTS_GENERIC_SHF10_Linear_Rail_Mount:2
- Równoległy:60 [Flush] (-3.5 mm): COTS_GENERIC_20x40mm_alu_extrusion_560mm:1 ↔ COTS_GENERIC_SHF10_Linear_Rail_Mount:1
- Zestawiający:59 [Mate]: COTS_GENERIC_SHF10_Linear_Rail_Mount:3 ↔ CUT_STEEL_10mmx457mm_Linear_Shaft:2
- Równoległy:61 [Flush] (-3.5 mm): COTS_GENERIC_20x40mm_alu_extrusion_560mm:3 ↔ COTS_GENERIC_SHF10_Linear_Rail_Mount:3
- Zestawiający:60 [Mate]: COTS_GENERIC_SHF10_Linear_Rail_Mount:4 ↔ CUT_STEEL_10mmx457mm_Linear_Shaft:1
- Równoległy:62 [Flush] (-3.5 mm): COTS_GENERIC_20x40mm_alu_extrusion_560mm:3 ↔ COTS_GENERIC_SHF10_Linear_Rail_Mount:4
- Zestawiający:61 [Mate] (1 mm): COTS_GENERIC_20x40mm_alu_extrusion_560mm:1 ↔ CUT_STEEL_10mmx457mm_Linear_Shaft:1
- Zestawiający:62 [Mate] (1 mm): COTS_GENERIC_20x40mm_alu_extrusion_560mm:1 ↔ CUT_STEEL_10mmx457mm_Linear_Shaft:2
- Zestawiający:63 [Mate] (215 mm): CUT_STEEL_10mmx457mm_Linear_Shaft:1 ↔ CUT_STEEL_10mmx457mm_Linear_Shaft:2
- Zestawiający:64 [Mate] (145 mm): COTS_GENERIC_20x40mm_alu_extrusion_460mm:2 ↔ CUT_STEEL_10mmx457mm_Linear_Shaft:2
- Zestawiający:65 [Mate]: CUT_STEEL_10mmx457mm_Linear_Shaft:2 ↔ COTS_GENERIC_LM10UU_10mm_Linear_Bearing:2
- Zestawiający:66 [Mate]: CUT_STEEL_10mmx457mm_Linear_Shaft:2 ↔ COTS_GENERIC_LM10UU_10mm_Linear_Bearing:1
- Zestawiający:67 [Mate]: CUT_STEEL_10mmx457mm_Linear_Shaft:1 ↔ COTS_GENERIC_LM10UU_10mm_Linear_Bearing:3
- Zestawiający:68 [Mate]: CUT_STEEL_10mmx457mm_Linear_Shaft:1 ↔ COTS_GENERIC_LM10UU_10mm_Linear_Bearing:4
- Zestawiający:71 [Mate] (-16.5 mm): CUT_STEEL_10mmx457mm_Linear_Shaft:1 ↔ LCBN_STEEL_3mm_Y_Axis_Heatbed_Baseplate:1
- Zestawiający:72 [Mate] (-16.5 mm): CUT_STEEL_10mmx457mm_Linear_Shaft:2 ↔ LCBN_STEEL_3mm_Y_Axis_Heatbed_Baseplate:1
- Zestawiający:73 [Mate] (5 mm): LCBN_STEEL_3mm_Y_Axis_Heatbed_Baseplate:1 ↔ CNCM_ALU_6mm_Heatbed:1
- Równoległy:63 [Flush] (0.5 mm): LCBN_STEEL_3mm_Y_Axis_Heatbed_Baseplate:1 ↔ CNCM_ALU_6mm_Heatbed:1
- Równoległy:64 [Flush] (40 mm): LCBN_STEEL_3mm_Y_Axis_Heatbed_Baseplate:1 ↔ CNCM_ALU_6mm_Heatbed:1
- Równoległy:65 [Flush]: COTS_GENERIC_SMA12GUU_Linear_Bearing_Block:2 ↔ COTS_GENERIC_SMA12GUU_Linear_Bearing_Block:4
- Równoległy:66 [Flush]: COTS_GENERIC_SMA12GUU_Linear_Bearing_Block:1 ↔ COTS_GENERIC_SMA12GUU_Linear_Bearing_Block:3
- Równoległy:67 [Flush]: COTS_GENERIC_SMA12GUU_Linear_Bearing_Block:1 ↔ COTS_GENERIC_SMA12GUU_Linear_Bearing_Block:2
- Zestawiający:76 [Mate] (6 mm): COTS_GENERIC_20x40mm_alu_extrusion_560mm:1 ↔ LCBN_ALU_2mm_Y_Axis_Motor_Mount:1
- Zestawiający:77 [Mate] (4 mm): LCBN_ALU_2mm_Y_Axis_Motor_Mount:1 ↔ COTS_GENERIC_NEMA23_Stepper_Motor:1
- Zestawiający:78 [Mate]: LCBN_ALU_2mm_Y_Axis_Motor_Mount:1 ↔ COTS_GENERIC_NEMA23_Stepper_Motor:1
- Równoległy:68 [Flush] (-1.85 mm): LCBN_ALU_2mm_Y_Axis_Motor_Mount:1 ↔ COTS_GENERIC_NEMA23_Stepper_Motor:1
- Zestawiający:79 [Mate]: COTS_GENERIC_20x40mm_alu_extrusion_560mm:3 ↔ 3DP_ABS_Feet:1
- Równoległy:69 [Flush]: COTS_GENERIC_20x40mm_alu_extrusion_460mm:1 ↔ 3DP_ABS_Feet:1
- Równoległy:70 [Flush]: COTS_GENERIC_20x40mm_alu_extrusion_560mm:3 ↔ 3DP_ABS_Feet:1
- Zestawiający:80 [Mate]: COTS_GENERIC_20x40mm_alu_extrusion_560mm:3 ↔ 3DP_ABS_Feet:3
- Równoległy:71 [Flush]: COTS_GENERIC_20x40mm_alu_extrusion_460mm:2 ↔ 3DP_ABS_Feet:3
- Równoległy:72 [Flush]: COTS_GENERIC_20x40mm_alu_extrusion_560mm:1 ↔ 3DP_ABS_Feet:3
- Zestawiający:81 [Mate]: COTS_GENERIC_20x40mm_alu_extrusion_560mm:3 ↔ 3DP_ABS_Feet_MIR:1
- Równoległy:73 [Flush]: COTS_GENERIC_20x40mm_alu_extrusion_460mm:2 ↔ 3DP_ABS_Feet_MIR:1
- Równoległy:74 [Flush]: COTS_GENERIC_20x40mm_alu_extrusion_560mm:3 ↔ 3DP_ABS_Feet_MIR:1
- Zestawiający:82 [Mate]: COTS_GENERIC_20x40mm_alu_extrusion_560mm:1 ↔ 3DP_ABS_Feet_MIR:2
- Równoległy:75 [Flush]: COTS_GENERIC_20x40mm_alu_extrusion_560mm:1 ↔ 3DP_ABS_Feet_MIR:2
- Równoległy:76 [Flush]: COTS_GENERIC_20x40mm_alu_extrusion_460mm:1 ↔ 3DP_ABS_Feet_MIR:2
- Równoległy:79 [Flush]: COTS_GENERIC_SMA12GUU_Linear_Bearing_Block:1 ↔ COTS_GENERIC_SMA12GUU_Linear_Bearing_Block:2
- Równoległy:80 [Flush]: COTS_GENERIC_SMA12GUU_Linear_Bearing_Block:3 ↔ COTS_GENERIC_SMA12GUU_Linear_Bearing_Block:4
- Zestawiający:84 [Mate]: COTS_GENERIC_20x40mm_alu_extrusion_460mm:3 ↔ 3DP_ABS_Z_Axis_Endstop_Mount:1
- Równoległy:81 [Flush]: COTS_GENERIC_20x40mm_alu_extrusion_460mm:3 ↔ 3DP_ABS_Z_Axis_Endstop_Mount:1
- Zestawiający:85 [Mate]: 3DP_ABS_Z_Axis_Endstop_Mount:1 ↔ COTS_GENERIC_Endstop:3
- Równoległy:82 [Flush]: 3DP_ABS_Z_Axis_Endstop_Mount:1 ↔ COTS_GENERIC_Endstop:3
- Równoległy:83 [Flush]: 3DP_ABS_Z_Axis_Endstop_Mount:1 ↔ COTS_GENERIC_Endstop:3
- Zestawiający:86 [Mate]: COTS_GENERIC_20x40mm_alu_extrusion_560mm:3 ↔ CNCM_ALU_3mm_Y_Axis_Idler_Stiffener_Side:1
- Zestawiający:87 [Mate]: COTS_GENERIC_20x40mm_alu_extrusion_560mm:3 ↔ CNCM_ALU_3mm_Y_Axis_Idler_Stiffener_Side:2
- Równoległy:84 [Flush]: COTS_GENERIC_20x40mm_alu_extrusion_560mm:3 ↔ CNCM_ALU_3mm_Y_Axis_Idler_Stiffener_Side:1
- Równoległy:85 [Flush]: COTS_GENERIC_20x40mm_alu_extrusion_560mm:3 ↔ CNCM_ALU_3mm_Y_Axis_Idler_Stiffener_Side:2
- Zestawiający:88 [Mate]: CNCM_ALU_3mm_Y_Axis_Idler_Stiffener_Side:1 ↔ LCBN_ALU_3mm_Y_Axis_Idler_Stiffener_Top:1
- Równoległy:86 [Flush]: CNCM_ALU_3mm_Y_Axis_Idler_Stiffener_Side:1 ↔ LCBN_ALU_3mm_Y_Axis_Idler_Stiffener_Top:1
- Zestawiający:89 [Mate]: CNCM_ALU_3mm_Y_Axis_Idler_Stiffener_Side:1 ↔ LCBN_ALU_3mm_Y_Axis_Idler_Stiffener_Top:1
- Zestawiający:90 [Mate]: CNCM_ALU_3mm_Y_Axis_Idler_Stiffener_Side:2 ↔ LCBN_ALU_3mm_Y_Axis_Idler_Stiffener_Top:1
- Zestawiający:94 [Mate]: COTS_GENERIC_20x40mm_alu_extrusion_560mm:1 ↔ 3DP_ABS_Y_Axis_Endstop_Mount:1
- Równoległy:89 [Flush]: COTS_GENERIC_20x40mm_alu_extrusion_560mm:1 ↔ 3DP_ABS_Y_Axis_Endstop_Mount:1
- Zestawiający:95 [Mate]: COTS_GENERIC_Endstop:1 ↔ 3DP_ABS_Y_Axis_Endstop_Mount:1
- Równoległy:90 [Flush]: COTS_GENERIC_Endstop:1 ↔ 3DP_ABS_Y_Axis_Endstop_Mount:1
- Równoległy:91 [Flush]: COTS_GENERIC_Endstop:1 ↔ 3DP_ABS_Y_Axis_Endstop_Mount:1
- Zestawiający:98 [Mate]: COTS_GENERIC_Bearing_12x5x5:1 ↔ COTS_GENERIC_Bearing_12x5x5:2
- Równoległy:92 [Flush] (249.5 mm): COTS_GENERIC_20x40mm_alu_extrusion_560mm:1 ↔ LCBN_ALU_2mm_Y_Axis_Motor_Mount:1